# Autodesk Inventor assembly: C-SCNPAW8-8
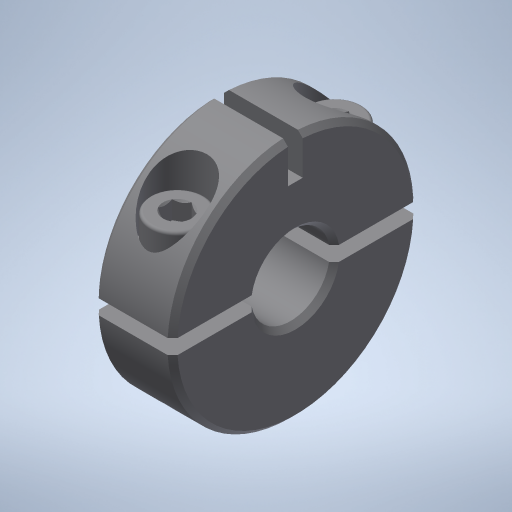
[picture p0: Inventor's stored thumbnail of the model, 512x512]
Saved by Autodesk Inventor 2024 (Build 280153020, 153B)
## iProperties
Created: 2023-10-03
Part Number: C-SCNPAW8-8
Catalog Web Link: www.cadenas.de
Description: C-SCNPAW-Economy Shaft Collars - Split
Vendor: MISUMI
Document SubType Name: Assembly
Designer: psAdmin
Manufacturer: MISUMI
Mass: 3.09963 g
Surface Area: 25.8765 cm^2
Volume: 3.09963 cm^3
Density: 1 g/cm^3
Category: PARTsolutions
Company: MISUMI
PSOL_IDENT_0: {$CADENAS_DATA/23d-libs/misumi/metric/03_set_collars/c_scnpaw_asmtab.prj},180 {VTYP=3D},{STYP=ASSTAB
PSOL_IDENT_1: },{NB=C-SCNPAW8-8},{LINA=C-SCNPAW8-8},{NN=C-SCNPAW},{DATE=12.09.2022 02:04:29},{GEOMDATE=08.03.2021
PSOL_IDENT_2: 12:07:16},{VERSION=},{LINEID=20},{WBVAR=B},{WBNUMERIC=B}  {NB=C-SCNPAW8-8},{LINA=C-SCNPAW8-8},{KT=DU
PSOL_IDENT_3: MMY},{PN=C-SCNPAW8-8},{D=8},{B=8},{BALG=8,10},{D1=25},{M1=M3},{M=3},{DD=3.4},{H=6.0},{W=1.5},{X=8.0}
PSOL_IDENT_4: ,{Y=5},{C=0.5},{L=10},{HH=4.0},{PPATH=c_scnpaw/c_scnpaw_asmtpl.prj}
NB: C-SCNPAW8-8
NN: C-SCNPAW
NT: Economy Shaft Collars - Split
NBSYN: $PN.
LINA: C-SCNPAW8-8
CATALOG: Misumi
PN: C-SCNPAW8-8
D: 8
B: 8
D1: 25
M1: M3
DD: 3.4
H: 6
W: 1.5
X: 8
Y: 5
SUPPLIER: MISUMI
ARTICLENO: C-SCNPAW8-8
BOMINFO: C-SCNPAW8-8
CREATOR: CADENAS GmbH
Title: C-SCNPAW8-8
Author: Cadenas PARTsolutions
Comments: Economy Shaft Collars - Split
## Documents named in this file (4)
- C:\Users\ryogo\OneDrive - Kyushu University\KURT_工房共有\2023~2024\ハード\CAD\2024NHK\000_parts\セットカラー\AIS2024\C-SCNPAW8-8.iam
- C:\Users\ryogo\OneDrive - Kyushu University\KURT_工房共有\2023~2024\ハード\CAD\2024NHK\000_parts\セットカラー\AIS2024\C-SCNPAW8-8_1.ipt
- C:\Users\ryogo\OneDrive - Kyushu University\KURT_工房共有\2023~2024\ハード\CAD\2024NHK\000_parts\セットカラー\AIS2024\C-SCNPAW8-8_2.ipt
- C:\Users\ryogo\OneDrive - Kyushu University\KURT_工房共有\2023~2024\ハード\CAD\2024NHK\000_parts\セットカラー\AIS2024\Slotted head cap screw ISO 4762 - M3x10.ipt
## Components (4 placed, 3 different names)
1. C-SCNPAW8-8_1:1 — to_body_XY@1 <-> to_body_XY@2, to_body_Z@1 <-> to_body_Z@2, to_body_YZ@1 <-> to_body_YZ@2, to_bolt_1_XY@1 <-> IP1_XY@3, to_bolt_1_Z@1 <-> IP1_Z@3, to_bolt_1_YZ@1 <-> IP1_YZ@3, to_bolt_2_XY@1 <-> IP1_XY@4, to_bolt_2_Z@1 <-> IP1_Z@4, to_bolt_2_YZ@1 <-> IP1_YZ@4
2. C-SCNPAW8-8_2:1 — to_body_XY@1 <-> to_body_XY@2, to_body_Z@1 <-> to_body_Z@2, to_body_YZ@1 <-> to_body_YZ@2
3. Slotted head cap screw ISO 4762 - M3x10:1 — to_bolt_1_XY@1 <-> IP1_XY@3, to_bolt_1_Z@1 <-> IP1_Z@3, to_bolt_1_YZ@1 <-> IP1_YZ@3
4. Slotted head cap screw ISO 4762 - M3x10:2 — to_bolt_2_XY@1 <-> IP1_XY@4, to_bolt_2_Z@1 <-> IP1_Z@4, to_bolt_2_YZ@1 <-> IP1_YZ@4
## Relationships (9: Mate 6, Angle 3)
- to_body_XY@1 <-> to_body_XY@2 [Mate]: C-SCNPAW8-8_1:1 ↔ C-SCNPAW8-8_2:1
- to_body_Z@1 <-> to_body_Z@2 [Mate]: C-SCNPAW8-8_1:1 ↔ C-SCNPAW8-8_2:1
- to_body_YZ@1 <-> to_body_YZ@2 [Angle] (0 deg): C-SCNPAW8-8_1:1 ↔ C-SCNPAW8-8_2:1
- to_bolt_1_XY@1 <-> IP1_XY@3 [Mate]: C-SCNPAW8-8_1:1 ↔ Slotted head cap screw ISO 4762 - M3x10:1
- to_bolt_1_Z@1 <-> IP1_Z@3 [Mate]: C-SCNPAW8-8_1:1 ↔ Slotted head cap screw ISO 4762 - M3x10:1
- to_bolt_1_YZ@1 <-> IP1_YZ@3 [Angle] (0 deg): C-SCNPAW8-8_1:1 ↔ Slotted head cap screw ISO 4762 - M3x10:1
- to_bolt_2_XY@1 <-> IP1_XY@4 [Mate]: C-SCNPAW8-8_1:1 ↔ Slotted head cap screw ISO 4762 - M3x10:2
- to_bolt_2_Z@1 <-> IP1_Z@4 [Mate]: C-SCNPAW8-8_1:1 ↔ Slotted head cap screw ISO 4762 - M3x10:2
- to_bolt_2_YZ@1 <-> IP1_YZ@4 [Angle] (0 deg): C-SCNPAW8-8_1:1 ↔ Slotted head cap screw ISO 4762 - M3x10:2
